# Autodesk Inventor assembly: PR01_assembly
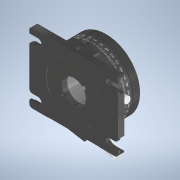
[picture p0: Inventor's stored thumbnail of the model, 180x180]
Saved by Autodesk Inventor 2021 (Build 250183000, 183)
## iProperties
Created: 2021-02-03
Part Number: PR01_assembly
Document SubType Name: Assembly
Designer: dsdan
Author: dsdan
## Documents named in this file (3)
- E:\OneDrive - Imperial College London\DragonVision_DanielKo\Instrumentation\Ephys_rig_2021\PR01_assembly.iam
- E:\OneDrive - Imperial College London\DragonVision_DanielKo\Instrumentation\Ephys_rig_2021\Imported Components\PR01A_M-Solidworks\PR01A_M-Solidworks.ipt
- E:\OneDrive - Imperial College London\DragonVision_DanielKo\Instrumentation\Ephys_rig_2021\Imported Components\PR01_M-Solidworks.ipt
## Components (2 placed, 2 different names)
1. PR01A_M-Solidworks:1 — Mate:1, Mate:2, Mate:3
2. PR01_M-Solidworks:1 — Mate:1, Mate:2, Mate:3
## Relationships (3: Mate 3)
- Mate:1: PR01A_M-Solidworks:1 ↔ PR01_M-Solidworks:1
- Mate:2: PR01A_M-Solidworks:1 ↔ PR01_M-Solidworks:1
- Mate:3: PR01A_M-Solidworks:1 ↔ PR01_M-Solidworks:1
